# Autodesk Inventor assembly: ExtruderAssem
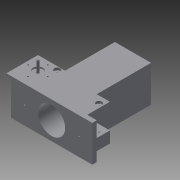
[picture p0: Inventor's stored thumbnail of the model, 180x180]
Saved by Autodesk Inventor 2015 SP2 (Build 190223200, 223)
## iProperties
Created: 2016-03-01
Part Number: ExtruderAssem
Document SubType Name: Assembly
Designer: marc
Author: marc
## Documents named in this file (3)
- C:\Users\marc\Documents\GitHub\Prusa_i3\Extruder\BeltDesign\ExtruderAssem.iam
- C:\Users\marc\Documents\GitHub\Prusa_i3\Extruder\BeltDesign\extruderBody.ipt
- C:\Users\marc\Documents\GitHub\Prusa_i3\Imported Components\NEMA 17 Stepper Motor Assembly\NEMA 17 Stepper Motor Assembly.iam
## Components (2 placed, 2 different names)
1. extruderBody:1 — Mate:1, Mate:2, Flush:1, Cylindrical:1, Mate:3, Cylindrical:2
2. NEMA 17 Stepper Motor Assembly:1 [sub-assembly] — Cylindrical:1, Mate:3, Cylindrical:2
## Relationships (6: Mate 3, CylindricalJoint 2, Flush 1)
- Mate:1: extruderBody:1
- Mate:2: extruderBody:1
- Flush:1: extruderBody:1
- Cylindrical:1: extruderBody:1 ↔ NEMA 17 Stepper Motor Assembly:1
- Mate:3: extruderBody:1 ↔ NEMA 17 Stepper Motor Assembly:1
- Cylindrical:2: extruderBody:1 ↔ NEMA 17 Stepper Motor Assembly:1
